# Autodesk Inventor assembly: ballCup
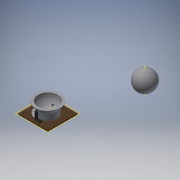
[picture p0: Inventor's stored thumbnail of the model, 180x180]
Saved by Autodesk Inventor 2016 (Build 200138000, 138)
## iProperties
Created: 2019-01-08
Part Number: ballCup
Document SubType Name: Assembly
Designer: harveylab
Author: harveylab
## Documents named in this file (8)
- C:\Users\harveylab\Documents\GitHub\mouseVR\Hardware\BallCupAssembly\ballCup.iam
- C:\Users\harveylab\Documents\GitHub\mouseVR\Hardware\BallCupAssembly\harvey_ballCup_ADNS9800_Vers1_1.ipt
- C:\Users\harveylab\Documents\GitHub\mouseVR\Hardware\BallCupAssembly\low_profile_noiseAttachment.ipt
- C:\Users\harveylab\Documents\GitHub\mouseVR\Hardware\BallCupAssembly\MB12.ipt
- C:\Users\harveylab\Documents\GitHub\mouseVR\Hardware\BallCupAssembly\PartBallCupAlignment.ipt
- C:\Users\harveylab\Documents\GitHub\mouseVR\Hardware\BallCupAssembly\vrRig_v0_8inBall.ipt
- C:\Users\harveylab\Documents\GitHub\mouseVR\Hardware\BallCupAssembly\UPH3-Solidworks.ipt
- C:\Users\harveylab\Documents\GitHub\mouseVR\Hardware\BallCupAssembly\TR2-Solidworks.ipt
## Components (9 placed, 7 different names)
1. harvey_ballCup_ADNS9800_Vers1_1:1 — Insert:4, Insert:5, Insert:6
2. low_profile_noiseAttachment:1 — Insert:3, Insert:4
3. MB12:1 — Insert:1, Insert:2, Mate:1, Mate:2
4. PartBallCupAlignment:1 — Insert:1, Insert:2, Insert:3
5. vrRig_v0_8inBall:1
6. UPH3-Solidworks:1 — Mate:2
7. UPH3-Solidworks:3 — Mate:1
8. TR2-Solidworks:1 — Insert:5
9. TR2-Solidworks:2 — Insert:6
## Relationships (8: Insert 6, Mate 2)
- Insert:1: MB12:1 ↔ PartBallCupAlignment:1
- Insert:2: MB12:1 ↔ PartBallCupAlignment:1
- Insert:3: low_profile_noiseAttachment:1 ↔ PartBallCupAlignment:1
- Insert:4 (-2.54 mm): harvey_ballCup_ADNS9800_Vers1_1:1 ↔ low_profile_noiseAttachment:1
- Mate:1: MB12:1 ↔ UPH3-Solidworks:3
- Mate:2: MB12:1 ↔ UPH3-Solidworks:1
- Insert:5: harvey_ballCup_ADNS9800_Vers1_1:1 ↔ TR2-Solidworks:1
- Insert:6: harvey_ballCup_ADNS9800_Vers1_1:1 ↔ TR2-Solidworks:2
